# Autodesk Inventor assembly: heater assembly
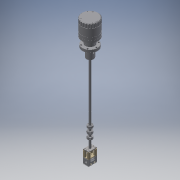
[picture p0: Inventor's stored thumbnail of the model, 180x180]
Saved by Autodesk Inventor 2018 (Build 220112000, 112)
## iProperties
Created: 2015-02-04
Part Number: heater assembly
Document SubType Name: Assembly
Designer: Pascal
Author: Pascal
## Documents named in this file (11)
- C:\Users\pnigge\Dropbox\UBC\Drawings\Heater\Heater drawings\heater assembly.iam
- C:\Users\pnigge\Dropbox\UBC\Drawings\Heater\Heater drawings\rotary feedthrough (MDC 670024) length extension.ipt
- C:\Users\pnigge\Dropbox\UBC\Drawings\Heater\Heater drawings\block.ipt
- C:\Users\pnigge\Dropbox\UBC\Drawings\Heater\Heater drawings\Shield_1.ipt
- C:\Users\pnigge\Dropbox\UBC\Drawings\Heater\Heater drawings\Shield_3.ipt
- C:\Users\pnigge\Dropbox\UBC\Drawings\Heater\Heater drawings\Shutter.ipt
- C:\Users\pnigge\Dropbox\UBC\Drawings\Heater\Heater drawings\ceramic washer.ipt
- C:\Users\pnigge\Dropbox\UBC\Drawings\Heater\Heater drawings\Shielding.ipt
- C:\Users\pnigge\Dropbox\UBC\Drawings\Heater\Heater drawings\Shielding side.ipt
- C:\Users\pnigge\Dropbox\UBC\Drawings\Heater\Heater drawings\alumina_standoff_LSP_ASO00110.ipt
- C:\Users\pnigge\Dropbox\UBC\Drawings\Heater\Heater drawings\9633T800_TWO-PIECE CLAMP-ON SHAFT COLLAR MOD.ipt
## Components (23 placed, 10 different names)
1. rotary feedthrough (MDC 670024) length extension:1 — Insert:1, Mate:45, Mate:47, Mate:49
2. block:2 — Mate:1, Flush:1, Flush:2, Mate:7, Mate:8, Mate:9, Flush:13, Flush:14, Mate:14, Mate:15, Mate:16, Mate:17, Mate:18, Mate:19, Mate:20, Mate:21, Flush:17, Flush:18, Mate:23, Mate:24, Mate:25, Mate:26, Mate:27, Mate:28, Mate:29, Mate:30, Flush:19, Mate:34, Flush:20
3. Shield_1:1 — Mate:1, Flush:1, Flush:2, Mate:35, Mate:36, Mate:37, Mate:38, Mate:39, Mate:40, Mate:41
4. Shield_3:1 — Insert:1, Mate:42, Mate:43, Mate:44, Mate:46, Angle:1, Angle:2, Angle:3
5. Shutter:1 — Mate:7, Mate:8, Mate:9
6. ceramic washer:1 — Mate:16, Mate:17, Mate:22
7. ceramic washer:2 — Mate:14, Mate:15
8. ceramic washer:3 — Mate:20, Mate:21
9. ceramic washer:4 — Mate:18, Mate:19
10. Shielding:1 — Mate:22, Flush:17, Flush:18
11. ceramic washer:5 — Mate:23, Mate:24, Mate:33
12. ceramic washer:6 — Mate:25, Mate:26
13. ceramic washer:7 — Mate:27, Mate:28, Mate:31, Mate:32
14. ceramic washer:8 — Mate:29, Mate:30
15. Shielding side:1 — Mate:31, Mate:32, Flush:19
16. Shielding side:2 — Mate:33, Mate:34, Flush:20
17. alumina_standoff_LSP_ASO00110:1 — Mate:40, Mate:41
18. alumina_standoff_LSP_ASO00110:2 — Mate:36, Mate:37, Mate:43, Mate:44
19. alumina_standoff_LSP_ASO00110:3 — Mate:35, Mate:42
20. alumina_standoff_LSP_ASO00110:4 — Mate:38, Mate:39
21. 9633T800_TWO-PIECE CLAMP-ON SHAFT COLLAR MOD:1 — Mate:45, Mate:46, Angle:1, Mate:48
22. 9633T800_TWO-PIECE CLAMP-ON SHAFT COLLAR MOD:2 — Mate:49, Mate:50, Angle:3
23. 9633T800_TWO-PIECE CLAMP-ON SHAFT COLLAR MOD:3 — Mate:47, Mate:48, Angle:2, Mate:50
## Relationships (53: Mate 41, Flush 8, Angle 3, Insert 1)
- Mate:1: block:2 ↔ Shield_1:1
- Flush:1: block:2 ↔ Shield_1:1
- Flush:2: block:2 ↔ Shield_1:1
- Insert:1: rotary feedthrough (MDC 670024) length extension:1 ↔ Shield_3:1
- Mate:7: block:2 ↔ Shutter:1
- Mate:8: block:2 ↔ Shutter:1
- Mate:9: block:2 ↔ Shutter:1
- Flush:13: block:2
- Flush:14: block:2
- Mate:14: block:2 ↔ ceramic washer:2
- Mate:15: block:2 ↔ ceramic washer:2
- Mate:16: block:2 ↔ ceramic washer:1
- Mate:17: block:2 ↔ ceramic washer:1
- Mate:18: block:2 ↔ ceramic washer:4
- Mate:19: block:2 ↔ ceramic washer:4
- Mate:20: block:2 ↔ ceramic washer:3
- Mate:21: block:2 ↔ ceramic washer:3
- Mate:22: ceramic washer:1 ↔ Shielding:1
- Flush:17: block:2 ↔ Shielding:1
- Flush:18: block:2 ↔ Shielding:1
- Mate:23: block:2 ↔ ceramic washer:5
- Mate:24: block:2 ↔ ceramic washer:5
- Mate:25: block:2 ↔ ceramic washer:6
- Mate:26: block:2 ↔ ceramic washer:6
- Mate:27: block:2 ↔ ceramic washer:7
- Mate:28: block:2 ↔ ceramic washer:7
- Mate:29: block:2 ↔ ceramic washer:8
- Mate:30: block:2 ↔ ceramic washer:8
- Mate:31: ceramic washer:7 ↔ Shielding side:1
- Mate:32: ceramic washer:7 ↔ Shielding side:1
- Flush:19: block:2 ↔ Shielding side:1
- Mate:33: ceramic washer:5 ↔ Shielding side:2
- Mate:34: block:2 ↔ Shielding side:2
- Flush:20: block:2 ↔ Shielding side:2
- Mate:35: Shield_1:1 ↔ alumina_standoff_LSP_ASO00110:3
- Mate:36: Shield_1:1 ↔ alumina_standoff_LSP_ASO00110:2
- Mate:37: Shield_1:1 ↔ alumina_standoff_LSP_ASO00110:2
- Mate:38: Shield_1:1 ↔ alumina_standoff_LSP_ASO00110:4
- Mate:39: Shield_1:1 ↔ alumina_standoff_LSP_ASO00110:4
- Mate:40: Shield_1:1 ↔ alumina_standoff_LSP_ASO00110:1
- Mate:41: Shield_1:1 ↔ alumina_standoff_LSP_ASO00110:1
- Mate:42: Shield_3:1 ↔ alumina_standoff_LSP_ASO00110:3
- Mate:43: Shield_3:1 ↔ alumina_standoff_LSP_ASO00110:2
- Mate:44: Shield_3:1 ↔ alumina_standoff_LSP_ASO00110:2
- Mate:45: rotary feedthrough (MDC 670024) length extension:1 ↔ 9633T800_TWO-PIECE CLAMP-ON SHAFT COLLAR MOD:1
- Mate:46 (38.1 mm): Shield_3:1 ↔ 9633T800_TWO-PIECE CLAMP-ON SHAFT COLLAR MOD:1
- Angle:1 (0 deg): Shield_3:1 ↔ 9633T800_TWO-PIECE CLAMP-ON SHAFT COLLAR MOD:1
- Mate:47: rotary feedthrough (MDC 670024) length extension:1 ↔ 9633T800_TWO-PIECE CLAMP-ON SHAFT COLLAR MOD:3
- Mate:48 (12.7 mm): 9633T800_TWO-PIECE CLAMP-ON SHAFT COLLAR MOD:1 ↔ 9633T800_TWO-PIECE CLAMP-ON SHAFT COLLAR MOD:3
- Angle:2 (0 deg): Shield_3:1 ↔ 9633T800_TWO-PIECE CLAMP-ON SHAFT COLLAR MOD:3
- Mate:49: rotary feedthrough (MDC 670024) length extension:1 ↔ 9633T800_TWO-PIECE CLAMP-ON SHAFT COLLAR MOD:2
- Mate:50 (12.7 mm): 9633T800_TWO-PIECE CLAMP-ON SHAFT COLLAR MOD:2 ↔ 9633T800_TWO-PIECE CLAMP-ON SHAFT COLLAR MOD:3
- Angle:3 (0 deg): Shield_3:1 ↔ 9633T800_TWO-PIECE CLAMP-ON SHAFT COLLAR MOD:2
